# Autodesk Inventor assembly: Ramabed
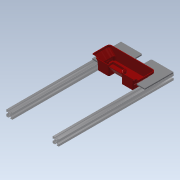
[picture p0: Inventor's stored thumbnail of the model, 180x180]
Saved by Autodesk Inventor 2022.1 (Build 261234020, 234B)
## iProperties
Created: 2022-07-22
Part Number: Ramabed
Document SubType Name: Assembly
Designer: Rama
Author: Rama
## Documents named in this file (6)
- C:\Users\Rama\Desktop\GitHub\Voron-2-Mods\Mandalaroseworks\BedPan\CAD\SRC\Mandala_BedPan.iam
- C:\Users\Rama\Desktop\GitHub\Voron-2-Mods\Mandalaroseworks\BedPan\CAD\SRC\Cover\Cover.ipt
- C:\Users\Rama\Desktop\GitHub\Voron-2-Mods\Mandalaroseworks\BedPan\CAD\SRC\Wagomount\Wagomount.ipt
- C:\Users\Rama\Desktop\GitHub\Voron-2-Mods\Mandalaroseworks\BedPan\CAD\SRC\Cableholder\Cableholder.ipt
- C:\Users\Rama\Desktop\RAMA_SBNG\ToolheadNEW\Bauteil1800.ipt
- C:\Users\Rama\Desktop\GitHub\Voron-2-Mods\Mandalaroseworks\BedPan\CAD\SRC\Bucket\Bucket_Offset.iam
## Components (6 placed, 5 different names)
1. Cover:1 — Passend:6, Passend:7, Fluchtend:4, Fluchtend:8, Passend:18, Passend:19
2. Wagomount:1 — Passend:1, Passend:2, Fluchtend:1, Passend:3, Passend:4, Passend:5, Passend:6, Passend:7, Fluchtend:4, Passend:10, Passend:11, Fluchtend:7
3. Cableholder:1 — Passend:3, Passend:4, Passend:5, Passend:17
4. Bauteil1800:1 — Fluchtend:5, Fluchtend:6, Passend:10
5. Bauteil1800:2 — Fluchtend:5, Fluchtend:6, Passend:11, Fluchtend:7, Fluchtend:8
6. Bucket_Offset:1 [sub-assembly] — Passend:17, Passend:18, Passend:19
## Relationships (18: Mate 12, Flush 6)
- Passend:1 [Mate]: Wagomount:1
- Passend:2 [Mate] (58 mm): Wagomount:1
- Fluchtend:1 [Flush]: Wagomount:1
- Passend:3 [Mate]: Wagomount:1 ↔ Cableholder:1
- Passend:4 [Mate]: Wagomount:1 ↔ Cableholder:1
- Passend:5 [Mate]: Wagomount:1 ↔ Cableholder:1
- Passend:6 [Mate]: Cover:1 ↔ Wagomount:1
- Passend:7 [Mate]: Cover:1 ↔ Wagomount:1
- Fluchtend:4 [Flush] (20 mm): Cover:1 ↔ Wagomount:1
- Fluchtend:5 [Flush]: Bauteil1800:1 ↔ Bauteil1800:2
- Fluchtend:6 [Flush]: Bauteil1800:1 ↔ Bauteil1800:2
- Passend:10 [Mate]: Wagomount:1 ↔ Bauteil1800:1
- Passend:11 [Mate]: Wagomount:1 ↔ Bauteil1800:2
- Fluchtend:7 [Flush]: Wagomount:1 ↔ Bauteil1800:2
- Fluchtend:8 [Flush]: Cover:1 ↔ Bauteil1800:2
- Passend:17 [Mate]: Cableholder:1 ↔ Bucket_Offset:1
- Passend:18 [Mate] (0.3 mm): Cover:1 ↔ Bucket_Offset:1
- Passend:19 [Mate] (0.3 mm): Cover:1 ↔ Bucket_Offset:1
